# Autodesk Inventor assembly: main assembly
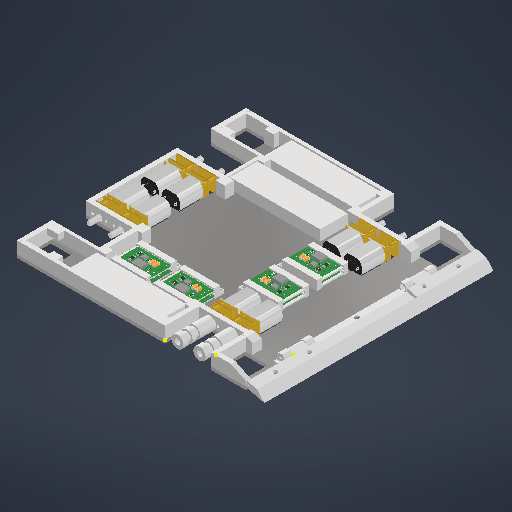
[picture p0: Inventor's stored thumbnail of the model, 512x512]
Saved by Autodesk Inventor 2026.2 (Build 302298010, 298A)
## iProperties
Created: 2026-04-27
Part Number: main assembly
Document SubType Name: Assembly
Designer: karol
Author: karol
## Documents named in this file (21)
- C:\Users\karol\Documents\GitHub\bolt\BOLT\cad\assembly\main assembly.iam
- C:\Users\karol\Documents\GitHub\bolt\BOLT\cad\ready parts\base.ipt
- C:\Users\karol\Documents\GitHub\bolt\BOLT\cad\ready parts\lewasciana.ipt
- C:\Users\karol\Documents\GitHub\bolt\BOLT\cad\ready parts\prawasciana.ipt
- C:\Users\karol\Documents\GitHub\bolt\BOLT\cad\ready parts\rmwall.ipt
- C:\Users\karol\Documents\GitHub\bolt\BOLT\cad\ready parts\lmwall.ipt
- C:\Users\karol\Documents\GitHub\bolt\BOLT\cad\ready parts\Pololu #2218 Micro Metal Gearmotor HP.ipt
- C:\Users\karol\Documents\GitHub\bolt\BOLT\cad\assembly\backmotors.iam
- C:\Users\karol\Documents\GitHub\bolt\BOLT\cad\ready parts\lewascianakoło.ipt
- C:\Users\karol\Documents\GitHub\bolt\BOLT\cad\ready parts\prawascianakolo.ipt
- C:\Users\karol\Documents\GitHub\bolt\BOLT\cad\ready parts\lfmw.ipt
- C:\Users\karol\Documents\GitHub\bolt\BOLT\cad\ready parts\rfmw.ipt
- C:\Users\karol\Documents\GitHub\bolt\BOLT\cad\ready parts\lipo.ipt
- C:\Users\karol\Documents\GitHub\bolt\BOLT\cad\assembly\plugassmbly.iam
- C:\Users\karol\Documents\GitHub\bolt\BOLT\cad\assembly\drvassembly.iam
- C:\Users\karol\Documents\GitHub\bolt\BOLT\cad\printing parts\rim-v1.ipt
- C:\Users\karol\Documents\GitHub\bolt\BOLT\cad\ready parts\zawias.ipt
- C:\Users\karol\Documents\GitHub\bolt\BOLT\cad\assembly\drvassemblylf.iam
- drvassemblylf.iam
- C:\Users\karol\Documents\GitHub\bolt\BOLT\cad\assembly\drvassemblyrf.iam
- drvassemblyrf.iam
## Components (25 placed, 18 different names)
1. base:1 — Zestawiające:1, Zestawiające:2, Zestawiające:3, Zestawiające:4, Zestawiające:5, Zestawiające:7, Zestawiające:15, Zestawiające:16, Zestawiające:17, Zestawiające:18, Zestawiające:21, Zestawiające:22, Zestawiające:23, Zestawiające:24, Zestawiające:28, Zestawiające:29, Zestawiające:30, Zestawiające:32, Zestawiające:33, Zestawiające:34, Zestawiające:35, Zestawiające:36, Zestawiające:37, Zestawiające:38, Zestawiające:39, Zestawiające:40, Zestawiające:41, Zestawiające:45, Zestawiające:47, Zestawiające:48, Zestawiające:62, Zestawiające:63, Zestawiające:64, Zestawiające:68, Zestawiające:73, Zestawiające:74, Zestawiające:75
2. lewasciana:1 — Zestawiające:1, Zestawiające:2, Zestawiające:46, Zestawiające:54, Zestawiające:55, Zestawiające:70, Zestawiające:71, Zestawiające:72
3. prawasciana:1 — Zestawiające:3, Zestawiające:4, Zestawiające:49, Zestawiające:56
4. rmwall:1 — Zestawiające:5, Zestawiające:48, Zestawiające:49, Zestawiające:50, Zestawiające:51, Zestawiające:79
5. lmwall:1 — Zestawiające:7, Zestawiające:52, Zestawiające:53, Zestawiające:54, Zestawiające:55, Równoległe:1, Równoległe:2, Zestawiające:61, Zestawiające:76
6. Pololu #2218 Micro Metal Gearmotor HP:3 — Zestawiające:17, Zestawiające:18
7. Pololu #2218 Micro Metal Gearmotor HP:4 — Zestawiające:15, Zestawiające:16
8. Pololu #2218 Micro Metal Gearmotor HP:7 — Zestawiające:21, Zestawiające:22
9. Pololu #2218 Micro Metal Gearmotor HP:8 — Zestawiające:23, Zestawiające:24, Zestawiające:60, Kątowe:1
10. lewascianakoło:1 — Zestawiające:32, Zestawiające:33, Zestawiające:69
11. prawascianakolo:1 — Zestawiające:28, Zestawiające:29, Zestawiające:30, Zestawiające:42, Zestawiające:43
12. backmotors:1 [sub-assembly] — Zestawiające:34, Zestawiające:35
13. lfmw:1 — Zestawiające:36, Zestawiające:37, Zestawiające:38, Zestawiające:52, Zestawiające:53, Zestawiające:77
14. rfmw:1 — Zestawiające:39, Zestawiające:40, Zestawiające:41, Zestawiające:50, Zestawiające:51, Zestawiające:78
15. lipo:2 — Zestawiające:46, Zestawiające:47
16. lipo:3 — Zestawiające:42, Zestawiające:43
17. lipo:4 — Zestawiające:45, Zestawiające:56
18. plugassmbly:1 [sub-assembly] — Zestawiające:65, Zestawiające:66, Zestawiające:67
19. drvassembly:1 [sub-assembly] — Zestawiające:68, Zestawiające:69, Zestawiające:70
20. drvassembly:2 [sub-assembly] — Zestawiające:71, Zestawiające:72, Zestawiające:73
21. rim-v1:1 — Równoległe:1, Równoległe:2
22. rim-v1:2 — Zestawiające:60, Kątowe:1, Zestawiające:61
23. zawias:1 — Zestawiające:62, Zestawiające:63, Zestawiające:64, Zestawiające:65, Zestawiające:66, Zestawiające:67
24. drvassemblylf:1 [sub-assembly] — Zestawiające:75, Zestawiające:78, Zestawiające:79
25. drvassemblyrf:3 [sub-assembly] — Zestawiające:74, Zestawiające:76, Zestawiające:77
## Relationships (64: Mate 61, Flush 2, Angle 1)
- Zestawiające:1 [Mate]: base:1 ↔ lewasciana:1
- Zestawiające:2 [Mate]: base:1 ↔ lewasciana:1
- Zestawiające:3 [Mate]: base:1 ↔ prawasciana:1
- Zestawiające:4 [Mate]: base:1 ↔ prawasciana:1
- Zestawiające:5 [Mate]: base:1 ↔ rmwall:1
- Zestawiające:7 [Mate]: base:1 ↔ lmwall:1
- Zestawiające:15 [Mate]: base:1 ↔ Pololu #2218 Micro Metal Gearmotor HP:4
- Zestawiające:16 [Mate]: base:1 ↔ Pololu #2218 Micro Metal Gearmotor HP:4
- Zestawiające:17 [Mate]: base:1 ↔ Pololu #2218 Micro Metal Gearmotor HP:3
- Zestawiające:18 [Mate]: base:1 ↔ Pololu #2218 Micro Metal Gearmotor HP:3
- Zestawiające:21 [Mate]: base:1 ↔ Pololu #2218 Micro Metal Gearmotor HP:7
- Zestawiające:22 [Mate]: base:1 ↔ Pololu #2218 Micro Metal Gearmotor HP:7
- Zestawiające:23 [Mate]: base:1 ↔ Pololu #2218 Micro Metal Gearmotor HP:8
- Zestawiające:24 [Mate]: base:1 ↔ Pololu #2218 Micro Metal Gearmotor HP:8
- Zestawiające:28 [Mate]: base:1 ↔ prawascianakolo:1
- Zestawiające:29 [Mate]: base:1 ↔ prawascianakolo:1
- Zestawiające:30 [Mate]: base:1 ↔ prawascianakolo:1
- Zestawiające:32 [Mate]: base:1 ↔ lewascianakoło:1
- Zestawiające:33 [Mate]: base:1 ↔ lewascianakoło:1
- Zestawiające:34 [Mate]: base:1 ↔ backmotors:1
- Zestawiające:35 [Mate]: base:1 ↔ backmotors:1
- Zestawiające:36 [Mate]: base:1 ↔ lfmw:1
- Zestawiające:37 [Mate]: base:1 ↔ lfmw:1
- Zestawiające:38 [Mate]: base:1 ↔ lfmw:1
- Zestawiające:39 [Mate]: base:1 ↔ rfmw:1
- Zestawiające:40 [Mate]: base:1 ↔ rfmw:1
- Zestawiające:41 [Mate]: base:1 ↔ rfmw:1
- Zestawiające:42 [Mate]: prawascianakolo:1 ↔ lipo:3
- Zestawiające:43 [Mate]: prawascianakolo:1 ↔ lipo:3
- Zestawiające:45 [Mate]: base:1 ↔ lipo:4
- Zestawiające:46 [Mate]: lewasciana:1 ↔ lipo:2
- Zestawiające:47 [Mate]: base:1 ↔ lipo:2
- Zestawiające:48 [Mate]: base:1 ↔ rmwall:1
- Zestawiające:49 [Mate]: prawasciana:1 ↔ rmwall:1
- Zestawiające:50 [Mate]: rmwall:1 ↔ rfmw:1
- Zestawiające:51 [Mate]: rmwall:1 ↔ rfmw:1
- Zestawiające:52 [Mate]: lmwall:1 ↔ lfmw:1
- Zestawiające:53 [Mate]: lmwall:1 ↔ lfmw:1
- Zestawiające:54 [Mate]: lewasciana:1 ↔ lmwall:1
- Zestawiające:55 [Mate]: lewasciana:1 ↔ lmwall:1
- Zestawiające:56 [Mate]: prawasciana:1 ↔ lipo:4
- Równoległe:1 [Flush]: lmwall:1 ↔ rim-v1:1
- Równoległe:2 [Flush] (0.5 mm): lmwall:1 ↔ rim-v1:1
- Zestawiające:60 [Mate]: Pololu #2218 Micro Metal Gearmotor HP:8 ↔ rim-v1:2
- Kątowe:1 [Angle] (180 deg): Pololu #2218 Micro Metal Gearmotor HP:8 ↔ rim-v1:2
- Zestawiające:61 [Mate]: lmwall:1 ↔ rim-v1:2
- Zestawiające:62 [Mate]: base:1 ↔ zawias:1
- Zestawiające:63 [Mate]: base:1 ↔ zawias:1
- Zestawiające:64 [Mate]: base:1 ↔ zawias:1
- Zestawiające:65 [Mate]: plugassmbly:1 ↔ zawias:1
- Zestawiające:66 [Mate]: plugassmbly:1 ↔ zawias:1
- Zestawiające:67 [Mate]: plugassmbly:1 ↔ zawias:1
- Zestawiające:68 [Mate]: base:1 ↔ drvassembly:1
- Zestawiające:69 [Mate] (5 mm): lewascianakoło:1 ↔ drvassembly:1
- Zestawiające:70 [Mate] (20 mm): lewasciana:1 ↔ drvassembly:1
- Zestawiające:71 [Mate] (4 mm): lewasciana:1 ↔ drvassembly:2
- Zestawiające:72 [Mate] (20 mm): lewasciana:1 ↔ drvassembly:2
- Zestawiające:73 [Mate]: base:1 ↔ drvassembly:2
- Zestawiające:74 [Mate]: base:1 ↔ drvassemblyrf:3
- Zestawiające:75 [Mate]: base:1 ↔ drvassemblylf:1
- Zestawiające:76 [Mate] (27 mm): lmwall:1 ↔ drvassemblyrf:3
- Zestawiające:77 [Mate] (8 mm): lfmw:1 ↔ drvassemblyrf:3
- Zestawiające:78 [Mate] (8 mm): rfmw:1 ↔ drvassemblylf:1
- Zestawiające:79 [Mate] (27 mm): rmwall:1 ↔ drvassemblylf:1
